# Autodesk Inventor assembly: fish_feeder
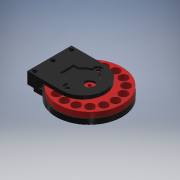
[picture p0: Inventor's stored thumbnail of the model, 180x180]
Saved by Autodesk Inventor 2019 (Build 230136000, 136)
## iProperties
Created: 2018-11-15
Part Number: fish_feeder
Document SubType Name: Assembly
Designer: chill
Author: chill
## Documents named in this file (5)
- C:\Users\chill\Desktop\fish_feeder.iam
- C:\Users\chill\Desktop\feeder_base.ipt
- C:\Users\chill\Desktop\feeder_motor_mount.ipt
- C:\Users\chill\Desktop\feeder_ring.ipt
- C:\Users\chill\Desktop\feeder_stack.ipt
## Components (4 placed, 4 different names)
1. feeder_base:1 — Mate:7, Mate:8, Mate:9, Mate:10, Mate:11, Mate:12, Mate:13
2. feeder_motor_mount:1 — Mate:1, Mate:2, Mate:3, Mate:4, Mate:5, Mate:6, Mate:8
3. feeder_ring:1 — Mate:1, Mate:2, Mate:13
4. feeder_stack:1 — Mate:3, Mate:4, Mate:5, Mate:6, Mate:7, Mate:9, Mate:10
## Relationships (13: Mate 13)
- Mate:1: feeder_motor_mount:1 ↔ feeder_ring:1
- Mate:2: feeder_motor_mount:1 ↔ feeder_ring:1
- Mate:3: feeder_motor_mount:1 ↔ feeder_stack:1
- Mate:4: feeder_motor_mount:1 ↔ feeder_stack:1
- Mate:5: feeder_motor_mount:1 ↔ feeder_stack:1
- Mate:6: feeder_motor_mount:1 ↔ feeder_stack:1
- Mate:7: feeder_base:1 ↔ feeder_stack:1
- Mate:8: feeder_base:1 ↔ feeder_motor_mount:1
- Mate:9: feeder_base:1 ↔ feeder_stack:1
- Mate:10: feeder_base:1 ↔ feeder_stack:1
- Mate:11: feeder_base:1
- Mate:12: feeder_base:1
- Mate:13: feeder_base:1 ↔ feeder_ring:1
